# Autodesk Inventor assembly: camera and mount block
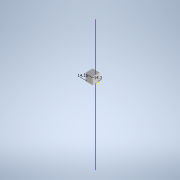
[picture p0: Inventor's stored thumbnail of the model, 180x180]
Saved by Autodesk Inventor 2020 (Build 240168000, 168)
## iProperties
Created: 2022-06-22
Part Number: camera and mount block
Document SubType Name: Assembly
Designer: Steven
Author: Steven
## Documents named in this file (3)
- Y:\FPV drone stuff\0 Street League\Frames\PB-Kauri-X\3D prints\35 mm canopy\work in progress prints\Camera mounts\predator nano\camera and mount block.iam
- Y:\FPV drone stuff\0 Street League\Frames\PB-Kauri-X\3D prints\35 mm canopy\work in progress prints\Camera mounts\predator nano\camera mount block.ipt
- Y:\FPV drone stuff\0 Street League\Frames\PB-Kauri-X\3D prints\35 mm canopy\work in progress prints\Camera mounts\predator nano\dummy camera.ipt
## Components (2 placed, 2 different names)
1. camera mount block:1 — Flush:1, Flush:2, Flush:3
2. dummy camera:1 — Flush:1, Flush:2, Flush:3
## Relationships (3: Flush 3)
- Flush:1 (2 mm): camera mount block:1 ↔ dummy camera:1
- Flush:2 (2 mm): camera mount block:1 ↔ dummy camera:1
- Flush:3: camera mount block:1 ↔ dummy camera:1
